# Autodesk Inventor assembly: robotetz
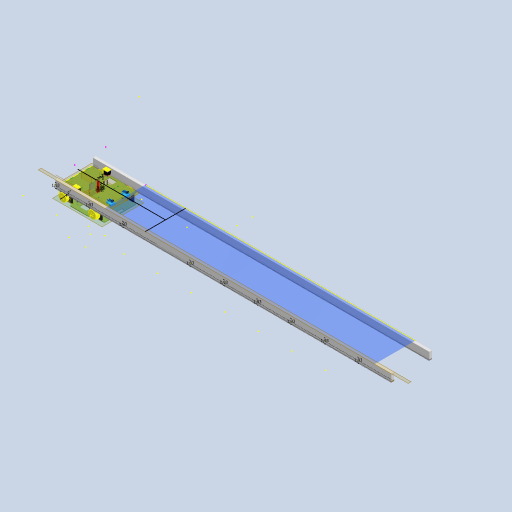
[picture p0: Inventor's stored thumbnail of the model, 512x512]
Saved by Autodesk Inventor 2024.2 (Build 282272000, 272)
## iProperties
Created: 2025-11-16
Part Number: robotetz
Document SubType Name: Assembly
Designer: katya_notebook
Mass: 10483.4 g
Surface Area: 22350.9 cm^2
Volume: 5372.63 cm^3
Density: 1.95127 g/cm^3
Author: katya_notebook
## Documents named in this file (49)
- C:\Users\91125\OneDrive\Рабочий стол\alletz\3д модель\etz\robotetz.iam
- C:\Users\91125\OneDrive\Рабочий стол\alletz\3д модель\полигон\полигон етз.iam
- C:\Users\91125\OneDrive\Рабочий стол\alletz\3д модель\Шестерня.ipt
- C:\Users\91125\OneDrive\Рабочий стол\alletz\3д модель\муфта.ipt
- C:\Users\91125\OneDrive\Рабочий стол\alletz\3д модель\Шестерня_MIR.ipt
- C:\Users\91125\OneDrive\Рабочий стол\alletz\3д модель\муфта_MIR.ipt
- C:\Users\91125\OneDrive\Рабочий стол\alletz\3д модель\мотор левая.iam
- C:\Users\91125\OneDrive\Рабочий стол\alletz\3д модель\мотор левая_MIR.iam
- C:\Users\91125\OneDrive\Рабочий стол\alletz\3д модель\нижняя пластина.ipt
- C:\Users\91125\OneDrive\Рабочий стол\alletz\3д модель\верхняя пластина.ipt
- C:\Users\91125\OneDrive\Рабочий стол\alletz\3д модель\крепление свободной шестерни.ipt
- C:\Users\91125\OneDrive\Рабочий стол\alletz\3д модель\Шестерня_MIR1.ipt
- C:\Users\91125\OneDrive\Рабочий стол\alletz\3д модель\Шестерня_MIR_MIR.ipt
- C:\Users\91125\OneDrive\Рабочий стол\alletz\3д модель\вал.ipt
- C:\Users\91125\OneDrive\Рабочий стол\alletz\3д модель\вал_MIR.ipt
- C:\Users\91125\OneDrive\Рабочий стол\alletz\3д модель\муфта_MIR1.ipt
- C:\Users\91125\OneDrive\Рабочий стол\alletz\3д модель\муфта_MIR_MIR.ipt
- C:\Users\91125\OneDrive\Рабочий стол\alletz\3д модель\цили.ipt
- C:\Users\91125\OneDrive\Рабочий стол\alletz\3д модель\подшипник.ipt
- C:\Users\91125\OneDrive\Рабочий стол\alletz\3д модель\верх штуки для подшипников.ipt
- C:\Users\91125\OneDrive\Рабочий стол\alletz\3д модель\крепление свободной шестерни_MIR.ipt
- C:\Users\91125\OneDrive\Рабочий стол\alletz\3д модель\цили_MIR2.ipt
- C:\Users\91125\OneDrive\Рабочий стол\alletz\3д модель\верх штуки для подшипников_MIR1.ipt
- C:\Users\91125\OneDrive\Рабочий стол\alletz\3д модель\подшипник_MIR.ipt
- C:\Users\91125\OneDrive\Рабочий стол\alletz\3д модель\магнит.ipt
- C:\Users\91125\OneDrive\Рабочий стол\alletz\3д модель\стопорное почти кольцо.ipt
- C:\Users\91125\OneDrive\Рабочий стол\alletz\3д модель\стопорное почти кольцо_MIR.ipt
- C:\Users\91125\OneDrive\Рабочий стол\alletz\3д модель\маркер.ipt
- C:\Users\91125\OneDrive\Рабочий стол\alletz\3д модель\шина.ipt
- C:\Users\91125\OneDrive\Рабочий стол\alletz\3д модель\диск.ipt
- C:\Users\91125\OneDrive\Рабочий стол\alletz\3д модель\шина_MIR1.ipt
- C:\Users\91125\OneDrive\Рабочий стол\alletz\3д модель\диск_MIR1.ipt
- C:\Users\91125\OneDrive\Рабочий стол\alletz\3д модель\вал_MIR_MIR.ipt
- C:\Users\91125\OneDrive\Рабочий стол\alletz\3д модель\муфта_MIR3.ipt
- C:\Users\91125\OneDrive\Рабочий стол\alletz\3д модель\энкодер.ipt
- C:\Users\91125\OneDrive\Рабочий стол\alletz\3д модель\крепление энкодера.ipt
- C:\Users\91125\OneDrive\Рабочий стол\alletz\3д модель\энкодер_MIR.ipt
- C:\Users\91125\OneDrive\Рабочий стол\alletz\3д модель\крепление энкодера_MIR.ipt
- C:\Users\91125\OneDrive\Рабочий стол\alletz\3д модель\Сервопривод с кареткой.iam
- C:\Users\91125\OneDrive\Рабочий стол\alletz\3д модель\магнит_MIR.ipt
- C:\Users\91125\OneDrive\Рабочий стол\alletz\3д модель\TCRT5000\TCRT5000.ipt
- C:\Users\91125\OneDrive\Рабочий стол\alletz\3д модель\крепление tcrt5000.ipt
- C:\Users\91125\OneDrive\Рабочий стол\alletz\3д модель\PROTOBOARD TOP.ipt
- C:\Users\91125\OneDrive\Рабочий стол\alletz\3д модель\стенка.ipt
- C:\Users\91125\OneDrive\Рабочий стол\alletz\3д модель\стенка 2.ipt
- C:\Users\91125\OneDrive\Рабочий стол\alletz\ETZ\ETZZ\ETZZ.ipt
- C:\Users\91125\OneDrive\Рабочий стол\alletz\3д модель\стойка для дисплея.ipt
- C:\Users\91125\OneDrive\Рабочий стол\alletz\3д модель\Holder 18650 (4 cell)_series_pink\Holder 18650 (4 cell)_series_pink.ipt
- C:\Users\91125\OneDrive\Рабочий стол\alletz\3д модель\проставка платы.ipt
## Components (57 placed, 48 different names)
1. полигон етз:1 [sub-assembly] — Заподлицо:1, Совмещение:1, Заподлицо:3, Заподлицо:8, Совмещение:11, Совмещение:42, Совмещение:43
2. нижняя пластина:1 — Заподлицо:9, Заподлицо:12, Совмещение:12, Совмещение:15, Совмещение:20, Совмещение:23, Совмещение:24, Совмещение:38, Совмещение:39, Заподлицо:33, Заподлицо:34, Заподлицо:35, Совмещение:45, Заподлицо:38, Заподлицо:40, С поворотом:4
3. верхняя пластина:1 — Заподлицо:10, Заподлицо:11, Заподлицо:13, Заподлицо:20, Совмещение:40, Заподлицо:31, Заподлицо:32, Заподлицо:43, Заподлицо:44, Совмещение:47, Заподлицо:47, Совмещение:48, Заподлицо:48, Заподлицо:49, Совмещение:49, Совмещение:50, Совмещение:51, Совмещение:52, Совмещение:53
4. маркер:1 — Совмещение:21, Совмещение:22
5. Сервопривод с кареткой:1 [sub-assembly] — Совмещение:38, Совмещение:39, С поворотом:4
6. TCRT5000:1 — Заподлицо:34, Совмещение:42
7. TCRT5000:2 — Заподлицо:35, Совмещение:43, Совмещение:46
8. крепление tcrt5000:1 — Заподлицо:33
9. PROTOBOARD TOP:1 — Совмещение:40, Заподлицо:31, Заподлицо:32
10. крепление tcrt5000:2 — Совмещение:45, Совмещение:46
11. стенка:1 — Заподлицо:38, Заподлицо:46
12. стенка 2:1 — Заподлицо:40
13. ETZZ:1 — Заподлицо:43, Заподлицо:44, Заподлицо:45, Совмещение:48
14. стойка для дисплея:1 — Заподлицо:45
15. Holder 18650 (4 cell)_series_pink:1 — Совмещение:47, Заподлицо:46, Заподлицо:47
16. проставка платы:1 — Заподлицо:48, Заподлицо:49
17. стенка 2:2 — Совмещение:50, Совмещение:51
18. стенка 2:3 — Совмещение:49
19. стенка 2:4 — Совмещение:52, Совмещение:53
20. Шестерня:1 — Заподлицо:1, Совмещение:1, С поворотом:1
21. муфта:1 — С поворотом:1, С поворотом:3
22. Шестерня_MIR:1 — С поворотом:2
23. муфта_MIR:1 — С поворотом:2
24. мотор левая:1 [sub-assembly] — С поворотом:3, Заподлицо:3, Заподлицо:9, Заподлицо:11
25. мотор левая_MIR:1 [sub-assembly] — Заподлицо:10
26. Шестерня_MIR1:1 — Заподлицо:26
27. Шестерня_MIR_MIR:1 — Заподлицо:14, Заподлицо:25, Заподлицо:39, Заподлицо:41, Заподлицо:42
28. вал:1 — Заподлицо:14, Цилиндрический:1, Заподлицо:25, Заподлицо:39, Заподлицо:41, Заподлицо:42
29. вал_MIR:1 — Цилиндрический:2, Цилиндрический:3, Заподлицо:26
30. муфта_MIR1:1
31. муфта_MIR_MIR:1
32. подшипник:1 — Совмещение:4, Совмещение:5
33. крепление свободной шестерни:1 — Заподлицо:12, Заподлицо:18
34. цили:1 — Заподлицо:21
35. верх штуки для подшипников:1 — Заподлицо:18, Заподлицо:19, Заподлицо:21
36. крепление свободной шестерни_MIR:1
37. цили_MIR2:1
38. верх штуки для подшипников_MIR1:1
39. подшипник_MIR:1 — Совмещение:8, Совмещение:9
40. стопорное почти кольцо:1 — Заподлицо:19, Заподлицо:20, Совмещение:5
41. стопорное почти кольцо:2 — Цилиндрический:1, Совмещение:4
42. стопорное почти кольцо_MIR:1 — Цилиндрический:3, Совмещение:9
43. стопорное почти кольцо_MIR:2 — Цилиндрический:2, Совмещение:8
44. магнит_MIR:1
45. вал_MIR:2 — Цилиндрический:4, Цилиндрический:5, Совмещение:28, Заподлицо:27
46. шина_MIR1:1 — Совмещение:17, Совмещение:18, Совмещение:19
47. диск_MIR1:1 — Совмещение:17, Совмещение:18, Совмещение:19, Совмещение:24, Совмещение:29, Заподлицо:28
48. муфта:3 — Цилиндрический:5, Совмещение:20
49. вал_MIR_MIR:1 — Цилиндрический:6, Совмещение:29, Заподлицо:28
50. муфта_MIR3:1 — Цилиндрический:6
51. шина:1 — Совмещение:11, Совмещение:12, Совмещение:13, Совмещение:14, Совмещение:16, Совмещение:25
52. диск:1 — Совмещение:13, Совмещение:14, Совмещение:15, Совмещение:16, Цилиндрический:4, Совмещение:23, Совмещение:28, Цилиндрический:7, Заподлицо:24, Заподлицо:27
53. энкодер:1 — Совмещение:25, Совмещение:30, Совмещение:31, Совмещение:32, Заподлицо:22, Совмещение:33
54. магнит:1 — Цилиндрический:7, Заподлицо:24
55. крепление энкодера:1 — Совмещение:32, Заподлицо:22, Совмещение:33
56. энкодер_MIR:1 — Совмещение:34, Совмещение:35, Совмещение:36, Заподлицо:23, Совмещение:37
57. крепление энкодера_MIR:1 — Совмещение:36, Заподлицо:23, Совмещение:37
## Relationships (96: Mate 44, Flush 40, CylindricalJoint 7, RevoluteJoint 4, WeldJoint 1)
- Заподлицо:1 [Flush]: полигон етз:1 ↔ Шестерня:1
- Совмещение:1 [Mate] (28 mm): полигон етз:1 ↔ Шестерня:1
- С поворотом:1 [RevoluteJoint]: Шестерня:1 ↔ муфта:1
- С поворотом:2 [RevoluteJoint]: Шестерня_MIR:1 ↔ муфта_MIR:1
- С поворотом:3 [RevoluteJoint]: муфта:1 ↔ мотор левая:1
- [WeldJoint]: муфта_MIR:1 ↔ мотор левая_MIR:1
- [Flush]: мотор левая:1 ↔ мотор левая_MIR:1
- Заподлицо:3 [Flush]: полигон етз:1 ↔ мотор левая:1
- [Flush]: мотор левая:1 ↔ мотор левая_MIR:1
- [Flush]: мотор левая:1 ↔ мотор левая_MIR:1
- Заподлицо:8 [Flush] (105 mm): полигон етз:1
- Заподлицо:9 [Flush]: нижняя пластина:1 ↔ мотор левая:1
- Заподлицо:10 [Flush]: верхняя пластина:1 ↔ мотор левая_MIR:1
- Заподлицо:11 [Flush]: верхняя пластина:1 ↔ мотор левая:1
- Заподлицо:12 [Flush]: нижняя пластина:1 ↔ крепление свободной шестерни:1
- Заподлицо:13 [Flush] (-135 mm): верхняя пластина:1
- Заподлицо:14 [Flush]: Шестерня_MIR_MIR:1 ↔ вал:1
- Заподлицо:18 [Flush]: крепление свободной шестерни:1 ↔ верх штуки для подшипников:1
- Заподлицо:19 [Flush]: верх штуки для подшипников:1 ↔ стопорное почти кольцо:1
- Заподлицо:20 [Flush]: верхняя пластина:1 ↔ стопорное почти кольцо:1
- Заподлицо:21 [Flush]: цили:1 ↔ верх штуки для подшипников:1
- Цилиндрический:1 [CylindricalJoint]: вал:1 ↔ стопорное почти кольцо:2
- Совмещение:4 [Mate]: подшипник:1 ↔ стопорное почти кольцо:2
- Совмещение:5 [Mate]: подшипник:1 ↔ стопорное почти кольцо:1
- Цилиндрический:2 [CylindricalJoint]: вал_MIR:1 ↔ стопорное почти кольцо_MIR:2
- Совмещение:8 [Mate]: подшипник_MIR:1 ↔ стопорное почти кольцо_MIR:2
- Цилиндрический:3 [CylindricalJoint]: вал_MIR:1 ↔ стопорное почти кольцо_MIR:1
- Совмещение:9 [Mate]: подшипник_MIR:1 ↔ стопорное почти кольцо_MIR:1
- Совмещение:11 [Mate] (15 mm): полигон етз:1 ↔ шина:1
- Совмещение:12 [Mate] (-100 mm): нижняя пластина:1 ↔ шина:1
- Совмещение:13 [Mate]: шина:1 ↔ диск:1
- Совмещение:14 [Mate]: шина:1 ↔ диск:1
- Совмещение:15 [Mate] (14 mm): нижняя пластина:1 ↔ диск:1
- Совмещение:16 [Mate]: шина:1 ↔ диск:1
- Совмещение:17 [Mate]: шина_MIR1:1 ↔ диск_MIR1:1
- Совмещение:18 [Mate]: шина_MIR1:1 ↔ диск_MIR1:1
- Совмещение:19 [Mate]: шина_MIR1:1 ↔ диск_MIR1:1
- Цилиндрический:4 [CylindricalJoint]: вал_MIR:2 ↔ диск:1
- Цилиндрический:5 [CylindricalJoint]: вал_MIR:2 ↔ муфта:3
- Совмещение:20 [Mate]: нижняя пластина:1 ↔ муфта:3
- Цилиндрический:6 [CylindricalJoint]: вал_MIR_MIR:1 ↔ муфта_MIR3:1
- Совмещение:21 [Mate]: маркер:1
- Совмещение:22 [Mate]: маркер:1
- Совмещение:23 [Mate] (5 mm): нижняя пластина:1 ↔ диск:1
- Совмещение:24 [Mate] (5 mm): нижняя пластина:1 ↔ диск_MIR1:1
- Совмещение:25 [Mate] (1.75 mm): шина:1 ↔ энкодер:1
- Совмещение:28 [Mate]: вал_MIR:2 ↔ диск:1
- Совмещение:29 [Mate]: диск_MIR1:1 ↔ вал_MIR_MIR:1
- Совмещение:30 [Mate] (-90 mm): энкодер:1
- Совмещение:31 [Mate] (35 mm): энкодер:1
- Совмещение:32 [Mate]: энкодер:1 ↔ крепление энкодера:1
- Заподлицо:22 [Flush]: энкодер:1 ↔ крепление энкодера:1
- Совмещение:33 [Mate]: энкодер:1 ↔ крепление энкодера:1
- Совмещение:34 [Mate] (35 mm): энкодер_MIR:1
- Совмещение:35 [Mate] (90 mm): энкодер_MIR:1
- Совмещение:36 [Mate]: энкодер_MIR:1 ↔ крепление энкодера_MIR:1
- Заподлицо:23 [Flush]: энкодер_MIR:1 ↔ крепление энкодера_MIR:1
- Совмещение:37 [Mate]: энкодер_MIR:1 ↔ крепление энкодера_MIR:1
- Цилиндрический:7 [CylindricalJoint]: диск:1 ↔ магнит:1
- Заподлицо:24 [Flush]: диск:1 ↔ магнит:1
- Совмещение:38 [Mate]: нижняя пластина:1 ↔ Сервопривод с кареткой:1
- Совмещение:39 [Mate]: нижняя пластина:1 ↔ Сервопривод с кареткой:1
- Заподлицо:25 [Flush]: Шестерня_MIR_MIR:1 ↔ вал:1
- Заподлицо:26 [Flush]: Шестерня_MIR1:1 ↔ вал_MIR:1
- Заподлицо:27 [Flush]: вал_MIR:2 ↔ диск:1
- Заподлицо:28 [Flush]: диск_MIR1:1 ↔ вал_MIR_MIR:1
- Совмещение:40 [Mate]: верхняя пластина:1 ↔ PROTOBOARD TOP:1
- Заподлицо:31 [Flush] (135 mm): верхняя пластина:1 ↔ PROTOBOARD TOP:1
- Заподлицо:32 [Flush] (12 mm): верхняя пластина:1 ↔ PROTOBOARD TOP:1
- Заподлицо:33 [Flush]: нижняя пластина:1 ↔ крепление tcrt5000:1
- Заподлицо:34 [Flush]: нижняя пластина:1 ↔ TCRT5000:1
- Заподлицо:35 [Flush]: нижняя пластина:1 ↔ TCRT5000:2
- Совмещение:42 [Mate] (53.5 mm): полигон етз:1 ↔ TCRT5000:1
- Совмещение:43 [Mate] (53.5 mm): полигон етз:1 ↔ TCRT5000:2
- Совмещение:45 [Mate]: нижняя пластина:1 ↔ крепление tcrt5000:2
- Совмещение:46 [Mate]: TCRT5000:2 ↔ крепление tcrt5000:2
- Заподлицо:38 [Flush]: нижняя пластина:1 ↔ стенка:1
- Заподлицо:39 [Flush]: Шестерня_MIR_MIR:1 ↔ вал:1
- Заподлицо:40 [Flush]: нижняя пластина:1 ↔ стенка 2:1
- Заподлицо:41 [Flush]: Шестерня_MIR_MIR:1 ↔ вал:1
- Заподлицо:42 [Flush]: Шестерня_MIR_MIR:1 ↔ вал:1
- Заподлицо:43 [Flush] (65 mm): верхняя пластина:1 ↔ ETZZ:1
- Заподлицо:44 [Flush] (25 mm): верхняя пластина:1 ↔ ETZZ:1
- Заподлицо:45 [Flush]: ETZZ:1 ↔ стойка для дисплея:1
- Совмещение:47 [Mate]: верхняя пластина:1 ↔ Holder 18650 (4 cell)_series_pink:1
- Заподлицо:46 [Flush] (15 mm): стенка:1 ↔ Holder 18650 (4 cell)_series_pink:1
- Заподлицо:47 [Flush] (60 mm): верхняя пластина:1 ↔ Holder 18650 (4 cell)_series_pink:1
- С поворотом:4 [RevoluteJoint]: нижняя пластина:1 ↔ Сервопривод с кареткой:1
- Совмещение:48 [Mate] (4 mm): верхняя пластина:1 ↔ ETZZ:1
- Заподлицо:48 [Flush]: верхняя пластина:1 ↔ проставка платы:1
- Заподлицо:49 [Flush]: верхняя пластина:1 ↔ проставка платы:1
- Совмещение:49 [Mate]: верхняя пластина:1 ↔ стенка 2:3
- Совмещение:50 [Mate]: верхняя пластина:1 ↔ стенка 2:2
- Совмещение:51 [Mate]: верхняя пластина:1 ↔ стенка 2:2
- Совмещение:52 [Mate]: верхняя пластина:1 ↔ стенка 2:4
- Совмещение:53 [Mate]: верхняя пластина:1 ↔ стенка 2:4
